# Autodesk Inventor assembly: full_vessel
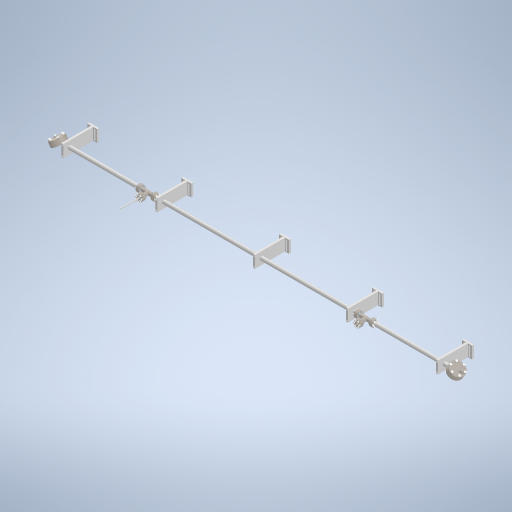
[picture p0: Inventor's stored thumbnail of the model, 512x512]
Saved by Autodesk Inventor 2024 (Build 280153000, 153)
## iProperties
Created: 2024-11-08
Part Number: full_vessel
Document SubType Name: Assembly
Designer: Andreas Weber
Author: Andreas Weber
## Documents named in this file (14)
- C:\Users\Andreas Weber\Desktop\Upload for Github\full_vessel.iam
- C:\Users\Andreas Weber\Desktop\Upload for Github\window_and_tee.iam
- C:\Users\Andreas Weber\Desktop\Upload for Github\tube_1m.ipt
- C:\Users\Andreas Weber\Desktop\Upload for Github\post.iam
- C:\Users\Andreas Weber\Desktop\Upload for Github\flange_camera_CF16.ipt
- C:\Users\Andreas Weber\Desktop\Upload for Github\flange_gas&pump.ipt
- C:\Users\Andreas Weber\Desktop\Upload for Github\Swagelok.ipt
- C:\Users\Andreas Weber\Desktop\Upload for Github\window_and_tee_MIR1.iam
- C:\Users\Andreas Weber\Desktop\Upload for Github\screw_ CF16.ipt
- C:\Users\Andreas Weber\Desktop\Upload for Github\screw_thread_CF40.ipt
- C:\Users\Andreas Weber\Desktop\Upload for Github\window_beam.ipt
- C:\Users\Andreas Weber\Desktop\Upload for Github\gasket_CF40.ipt
- C:\Users\Andreas Weber\Desktop\Upload for Github\gasket_CF16.ipt
- C:\Users\Andreas Weber\Desktop\Upload for Github\window_camera.ipt
## Components (70 placed, 13 different names)
1. window_and_tee:1 [sub-assembly] — Drehbar:1, Einfügen:2, Einfügen:3, Einfügen:6, Drehbar:2, Drehbar:17, Drehbar:18, Drehbar:19, Drehbar:20, Drehbar:21, Drehbar:22, Drehbar:23, Drehbar:24, Drehbar:25, Drehbar:26, Drehbar:27, Drehbar:28, Drehbar:47, Drehbar:48, Drehbar:49, Drehbar:50, Drehbar:51, Drehbar:52, Starr:1, Drehbar:53, Drehbar:56, Drehbar:57
2. tube_1m:1 — Drehbar:1, Einfügen:7
3. post:1 [sub-assembly]
4. post:2 [sub-assembly]
5. post:3 [sub-assembly] — Einfügen:2
6. post:4 [sub-assembly] — Einfügen:3
7. post:5 [sub-assembly] — Einfügen:6
8. flange_camera_CF16:1 — Drehbar:2, Drehbar:5, Drehbar:6, Drehbar:7, Drehbar:8, Drehbar:9, Drehbar:10, Drehbar:54, Drehbar:55
9. window_and_tee_MIR1:1 [sub-assembly] — Einfügen:7, Drehbar:3, Drehbar:29, Drehbar:30, Drehbar:31, Drehbar:32, Drehbar:33, Drehbar:34, Drehbar:35, Drehbar:36, Drehbar:37, Drehbar:38, Drehbar:39, Drehbar:40, Drehbar:41, Drehbar:42, Drehbar:43, Drehbar:44, Drehbar:45, Drehbar:46, Drehbar:58, Drehbar:59, Drehbar:62, Drehbar:63
10. flange_gas&pump:1 — Drehbar:3, Drehbar:4, Drehbar:11, Drehbar:12, Drehbar:13, Drehbar:14, Drehbar:15, Drehbar:16, Drehbar:60
11. Swagelok:1 — Drehbar:4
12. screw_ CF16:1 — Drehbar:8
13. screw_ CF16:2 — Drehbar:9
14. screw_ CF16:3 — Drehbar:10
15. screw_ CF16:4 — Drehbar:6
16. screw_ CF16:5 — Drehbar:5
17. screw_ CF16:6 — Drehbar:7
18. screw_ CF16:7 — Drehbar:11
19. screw_ CF16:8 — Drehbar:12
20. screw_ CF16:9 — Drehbar:13
21. screw_ CF16:10 — Drehbar:14
22. screw_ CF16:11 — Drehbar:15
23. screw_ CF16:12 — Drehbar:16
24. screw_ CF16:13 — Drehbar:17
25. screw_ CF16:14 — Drehbar:18
26. screw_ CF16:15 — Drehbar:19
27. screw_ CF16:16 — Drehbar:20
28. screw_ CF16:17 — Drehbar:21
29. screw_ CF16:18 — Drehbar:22
30. screw_ CF16:19 — Drehbar:24
31. screw_ CF16:20 — Drehbar:25
32. screw_ CF16:21 — Drehbar:26
33. screw_ CF16:22 — Drehbar:27
34. screw_ CF16:23 — Drehbar:28
35. screw_ CF16:24 — Drehbar:23
36. screw_ CF16:25 — Drehbar:30
37. screw_ CF16:26 — Drehbar:31
38. screw_ CF16:27 — Drehbar:32
39. screw_ CF16:28 — Drehbar:33
40. screw_ CF16:29 — Drehbar:34
41. screw_ CF16:30 — Drehbar:29
42. screw_ CF16:31 — Drehbar:35
43. screw_ CF16:32 — Drehbar:36
44. screw_ CF16:33 — Drehbar:37
45. screw_ CF16:34 — Drehbar:38
46. screw_ CF16:35 — Drehbar:39
47. screw_ CF16:36 — Drehbar:40
48. screw_thread_CF40:1 — Drehbar:42
49. screw_thread_CF40:2 — Drehbar:43
50. screw_thread_CF40:3 — Drehbar:44
51. screw_thread_CF40:4 — Drehbar:45
52. screw_thread_CF40:5 — Drehbar:46
53. screw_thread_CF40:6 — Drehbar:41
54. screw_thread_CF40:7 — Drehbar:47
55. screw_thread_CF40:8 — Drehbar:48
56. screw_thread_CF40:9 — Drehbar:49
57. screw_thread_CF40:10 — Drehbar:50
58. screw_thread_CF40:11 — Drehbar:51
59. screw_thread_CF40:12 — Drehbar:52
60. window_beam:1 — Starr:1
61. gasket_CF40:1 — Drehbar:53
62. gasket_CF16:1 — Drehbar:54
63. gasket_CF16:2 — Drehbar:56
64. gasket_CF16:3 — Drehbar:57
65. window_camera:1 — Drehbar:55
66. window_beam:2 — Drehbar:58
67. gasket_CF40:2 — Drehbar:59
68. gasket_CF16:4 — Drehbar:60
69. gasket_CF16:6 — Drehbar:62
70. gasket_CF16:7 — Drehbar:63
## Relationships (67: RevoluteJoint 62, Insert 4, WeldJoint 1)
- Drehbar:1 [RevoluteJoint]: window_and_tee:1 ↔ tube_1m:1
- Einfügen:2 [Insert] (-355 mm): window_and_tee:1 ↔ post:3
- Einfügen:3 [Insert] (20 mm): window_and_tee:1 ↔ post:4
- Einfügen:6 [Insert] (-492.65 mm): window_and_tee:1 ↔ post:5
- Drehbar:2 [RevoluteJoint]: window_and_tee:1 ↔ flange_camera_CF16:1
- Einfügen:7 [Insert]: tube_1m:1 ↔ window_and_tee_MIR1:1
- Drehbar:3 [RevoluteJoint]: window_and_tee_MIR1:1 ↔ flange_gas&pump:1
- Drehbar:4 [RevoluteJoint]: flange_gas&pump:1 ↔ Swagelok:1
- Drehbar:5 [RevoluteJoint]: flange_camera_CF16:1 ↔ screw_ CF16:5
- Drehbar:6 [RevoluteJoint]: flange_camera_CF16:1 ↔ screw_ CF16:4
- Drehbar:7 [RevoluteJoint]: flange_camera_CF16:1 ↔ screw_ CF16:6
- Drehbar:8 [RevoluteJoint]: flange_camera_CF16:1 ↔ screw_ CF16:1
- Drehbar:9 [RevoluteJoint]: flange_camera_CF16:1 ↔ screw_ CF16:2
- Drehbar:10 [RevoluteJoint]: flange_camera_CF16:1 ↔ screw_ CF16:3
- Drehbar:11 [RevoluteJoint]: flange_gas&pump:1 ↔ screw_ CF16:7
- Drehbar:12 [RevoluteJoint]: flange_gas&pump:1 ↔ screw_ CF16:8
- Drehbar:13 [RevoluteJoint]: flange_gas&pump:1 ↔ screw_ CF16:9
- Drehbar:14 [RevoluteJoint]: flange_gas&pump:1 ↔ screw_ CF16:10
- Drehbar:15 [RevoluteJoint]: flange_gas&pump:1 ↔ screw_ CF16:11
- Drehbar:16 [RevoluteJoint]: flange_gas&pump:1 ↔ screw_ CF16:12
- Drehbar:17 [RevoluteJoint]: window_and_tee:1 ↔ screw_ CF16:13
- Drehbar:18 [RevoluteJoint]: window_and_tee:1 ↔ screw_ CF16:14
- Drehbar:19 [RevoluteJoint]: window_and_tee:1 ↔ screw_ CF16:15
- Drehbar:20 [RevoluteJoint]: window_and_tee:1 ↔ screw_ CF16:16
- Drehbar:21 [RevoluteJoint]: window_and_tee:1 ↔ screw_ CF16:17
- Drehbar:22 [RevoluteJoint]: window_and_tee:1 ↔ screw_ CF16:18
- Drehbar:23 [RevoluteJoint]: window_and_tee:1 ↔ screw_ CF16:24
- Drehbar:24 [RevoluteJoint]: window_and_tee:1 ↔ screw_ CF16:19
- Drehbar:25 [RevoluteJoint]: window_and_tee:1 ↔ screw_ CF16:20
- Drehbar:26 [RevoluteJoint]: window_and_tee:1 ↔ screw_ CF16:21
- Drehbar:27 [RevoluteJoint]: window_and_tee:1 ↔ screw_ CF16:22
- Drehbar:28 [RevoluteJoint]: window_and_tee:1 ↔ screw_ CF16:23
- Drehbar:29 [RevoluteJoint]: window_and_tee_MIR1:1 ↔ screw_ CF16:30
- Drehbar:30 [RevoluteJoint]: window_and_tee_MIR1:1 ↔ screw_ CF16:25
- Drehbar:31 [RevoluteJoint]: window_and_tee_MIR1:1 ↔ screw_ CF16:26
- Drehbar:32 [RevoluteJoint]: window_and_tee_MIR1:1 ↔ screw_ CF16:27
- Drehbar:33 [RevoluteJoint]: window_and_tee_MIR1:1 ↔ screw_ CF16:28
- Drehbar:34 [RevoluteJoint]: window_and_tee_MIR1:1 ↔ screw_ CF16:29
- Drehbar:35 [RevoluteJoint]: window_and_tee_MIR1:1 ↔ screw_ CF16:31
- Drehbar:36 [RevoluteJoint]: window_and_tee_MIR1:1 ↔ screw_ CF16:32
- Drehbar:37 [RevoluteJoint]: window_and_tee_MIR1:1 ↔ screw_ CF16:33
- Drehbar:38 [RevoluteJoint]: window_and_tee_MIR1:1 ↔ screw_ CF16:34
- Drehbar:39 [RevoluteJoint]: window_and_tee_MIR1:1 ↔ screw_ CF16:35
- Drehbar:40 [RevoluteJoint]: window_and_tee_MIR1:1 ↔ screw_ CF16:36
- Drehbar:41 [RevoluteJoint]: window_and_tee_MIR1:1 ↔ screw_thread_CF40:6
- Drehbar:42 [RevoluteJoint]: window_and_tee_MIR1:1 ↔ screw_thread_CF40:1
- Drehbar:43 [RevoluteJoint]: window_and_tee_MIR1:1 ↔ screw_thread_CF40:2
- Drehbar:44 [RevoluteJoint]: window_and_tee_MIR1:1 ↔ screw_thread_CF40:3
- Drehbar:45 [RevoluteJoint]: window_and_tee_MIR1:1 ↔ screw_thread_CF40:4
- Drehbar:46 [RevoluteJoint]: window_and_tee_MIR1:1 ↔ screw_thread_CF40:5
- Drehbar:47 [RevoluteJoint]: window_and_tee:1 ↔ screw_thread_CF40:7
- Drehbar:48 [RevoluteJoint]: window_and_tee:1 ↔ screw_thread_CF40:8
- Drehbar:49 [RevoluteJoint]: window_and_tee:1 ↔ screw_thread_CF40:9
- Drehbar:50 [RevoluteJoint]: window_and_tee:1 ↔ screw_thread_CF40:10
- Drehbar:51 [RevoluteJoint]: window_and_tee:1 ↔ screw_thread_CF40:11
- Drehbar:52 [RevoluteJoint]: window_and_tee:1 ↔ screw_thread_CF40:12
- Starr:1 [WeldJoint]: window_and_tee:1 ↔ window_beam:1
- Drehbar:53 [RevoluteJoint]: window_and_tee:1 ↔ gasket_CF40:1
- Drehbar:54 [RevoluteJoint]: flange_camera_CF16:1 ↔ gasket_CF16:1
- Drehbar:55 [RevoluteJoint]: flange_camera_CF16:1 ↔ window_camera:1
- Drehbar:56 [RevoluteJoint]: window_and_tee:1 ↔ gasket_CF16:2
- Drehbar:57 [RevoluteJoint]: window_and_tee:1 ↔ gasket_CF16:3
- Drehbar:58 [RevoluteJoint]: window_and_tee_MIR1:1 ↔ window_beam:2
- Drehbar:59 [RevoluteJoint]: window_and_tee_MIR1:1 ↔ gasket_CF40:2
- Drehbar:60 [RevoluteJoint]: flange_gas&pump:1 ↔ gasket_CF16:4
- Drehbar:62 [RevoluteJoint]: window_and_tee_MIR1:1 ↔ gasket_CF16:6
- Drehbar:63 [RevoluteJoint]: window_and_tee_MIR1:1 ↔ gasket_CF16:7
